# Autodesk Inventor assembly: link_first
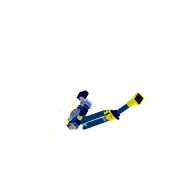
[picture p0: Inventor's stored thumbnail of the model, 180x180]
Saved by Autodesk Inventor 2020.5 (Build 245400000, 400)
## iProperties
Created: 2022-10-31
Part Number: link_first
Document SubType Name: Assembly
Designer: kanazawakotaro
Author: Administrator
## Documents named in this file (18)
- C:\Users\Administrator\Documents\kamuy2\kamuy2\link_first.iam
- C:\Users\Administrator\Documents\kamuy2\kamuy2\Parts\Part2_MIR_CPY_MIR.ipt
- C:\Users\Administrator\Documents\kamuy2\kamuy2\Parts\x-540_idle_MIR_CPY_MIR.ipt
- C:\Users\Administrator\Documents\kamuy2\kamuy2\Parts\GEABP1.0-32-10-A-12-KFC22-K3_Autodesk_Inventor_2020_20221101\AIS2020\GEABP1_0-32-10-A-12-KFC22-K3_MIR_CPY_MIR.iam
- C:\Users\Administrator\Documents\kamuy2\kamuy2\Parts\GEYK1.0-70-10-B-10K_Autodesk_Inventor_2020_20221114\AIS2020\GEYK1_0-70-10-B-10K_MIR_CPY_MIR.iam
- C:\Users\Administrator\Documents\kamuy2\kamuy2\Part16_MIR_CPY_MIR.ipt
- C:\Users\Administrator\Documents\kamuy2\kamuy2\Part1_MIR_CPY_MIR.ipt
- C:\Users\Administrator\Documents\kamuy2\kamuy2\Part13_MIR_CPY_MIR.ipt
- C:\Users\Administrator\Documents\kamuy2\kamuy2\Part17_MIR_CPY_MIR.ipt
- C:\Users\Administrator\Documents\kamuy2\kamuy2\Parts\SMYHF10_STEP_AP203AP214\SMYHF10_203_MIR_CPY_MIR.ipt
- C:\Users\Administrator\Documents\kamuy2\kamuy2\Parts\BGHK6800VV-30_Autodesk_Inventor_2020_20221102\AIS2020\BGHK6800VV-30_MIR_CPY_MIR.iam
- C:\Users\Administrator\Documents\kamuy2\kamuy2\Parts\XW540.N105.I101_MIR_CPY_MIR.ipt
- C:\Users\Administrator\Documents\kamuy2\kamuy2\Parts\NSFMKR10-67-KA22-A20_Autodesk_Inventor_2020_20221116\AIS2020\NSFMKR10-67-KA22-A20_MIR_CPY_MIR.iam
- C:\Users\Administrator\Documents\kamuy2\kamuy2\Parts\NSFMR10-37_Autodesk_Inventor_2020_20221116\AIS2020\NSFMR10-37(000_000)_MIR_CPY_MIR.iam
- C:\Users\Administrator\Documents\kamuy2\kamuy2\Parts\NSFMKRRA10-144-F3-S6-KA5-A18-KB108.5-B11_Autodesk_Inventor_2020_20221117\AIS2020\NSFMKRRA10-144-F3-S6-KA5-A18-KB108_5-B11_MIR_CPY_MIR.iam
- C:\Users\Administrator\Documents\kamuy2\kamuy2\LEG_MIR_MIR1_MIR.iam
- C:\Users\Administrator\Documents\foot3d.ipt
- C:\Users\Administrator\Documents\gom.ipt
## Components (27 placed, 17 different names)
1. Part2_MIR_CPY_MIR:1
2. x-540_idle_MIR_CPY_MIR:1 — メイト:51, メイト:50, フラッシュ:68, フラッシュ:66, フラッシュ:58, メイト:166, フラッシュ:103, メイト:256, メイト:39
3. GEABP1_0-32-10-A-12-KFC22-K3_MIR_CPY_MIR:1 [sub-assembly] — メイト:51, メイト:50, フラッシュ:20
4. GEYK1_0-70-10-B-10K_MIR_CPY_MIR:1 [sub-assembly] — フラッシュ:61, フラッシュ:136, メイト:248
5. x-540_idle_MIR_CPY_MIR:2 — フラッシュ:68, フラッシュ:66, フラッシュ:58, メイト:86, メイト:85, フラッシュ:100, メイト:183, メイト:180, メイト:179, メイト:178
6. GEABP1_0-32-10-A-12-KFC22-K3_MIR_CPY_MIR:2 [sub-assembly] — フラッシュ:61, メイト:86, メイト:85
7. Part16_MIR_CPY_MIR:1 — メイト:170
8. Part16_MIR_CPY_MIR:2 — メイト:171
9. Part1_MIR_CPY_MIR:1 — メイト:171, フラッシュ:100
10. Part1_MIR_CPY_MIR:2 — メイト:183, メイト:170, メイト:166, メイト:38, メイト:39
11. Part13_MIR_CPY_MIR:1 — フラッシュ:103, フラッシュ:108, フラッシュ:104, メイト:172, メイト:208
12. Part17_MIR_CPY_MIR:1 — フラッシュ:108, フラッシュ:104, メイト:172, フラッシュ:105, メイト:174, メイト:177
13. SMYHF10_203_MIR_CPY_MIR:1 — フラッシュ:105, メイト:174, メイト:254
14. GEYK1_0-70-10-B-10K_MIR_CPY_MIR:2 [sub-assembly] — メイト:177, メイト:65, メイト:207
15. Part13_MIR_CPY_MIR:2 — メイト:180, メイト:179, メイト:178, フラッシュ:110, メイト:194, メイト:214
16. SMYHF10_203_MIR_CPY_MIR:2 — メイト:187, メイト:185, メイト:213
17. Part17_MIR_CPY_MIR:2 — フラッシュ:110, メイト:194, メイト:187, メイト:185, メイト:211, メイト:215
18. BGHK6800VV-30_MIR_CPY_MIR:1 [sub-assembly] — メイト:65, フラッシュ:33, フラッシュ:32, メイト:205, メイト:209, フラッシュ:116, フラッシュ:115
19. GEABP1_0-32-10-A-12-KFC22-K3_MIR_CPY_MIR:3 [sub-assembly] — メイト:204, メイト:203
20. XW540.N105.I101_MIR_CPY_MIR:1 — フラッシュ:33, フラッシュ:32, メイト:205, メイト:204, メイト:203
21. NSFMKR10-67-KA22-A20_MIR_CPY_MIR:1 [sub-assembly] — メイト:254, メイト:209, メイト:208, メイト:207
22. BGHK6800VV-30_MIR_CPY_MIR:2 [sub-assembly] — メイト:211, フラッシュ:116, フラッシュ:115, メイト:212
23. NSFMR10-37(000_000)_MIR_CPY_MIR:1 [sub-assembly] — メイト:215, メイト:214, メイト:213, メイト:212
24. NSFMKRRA10-144-F3-S6-KA5-A18-KB108_5-B11_MIR_CPY_MIR:1 [sub-assembly] — メイト:256, フラッシュ:136, メイト:248, メイト:37, メイト:38
25. LEG_MIR_MIR1_MIR:1 [sub-assembly] — メイト:37, フラッシュ:20, メイト:42, メイト:43, フラッシュ:22
26. foot3d:1 — メイト:42, メイト:43, フラッシュ:22
27. gom:1
## Relationships (57: Mate 39, Flush 18)
- メイト:51 [Mate]: x-540_idle_MIR_CPY_MIR:1 ↔ GEABP1_0-32-10-A-12-KFC22-K3_MIR_CPY_MIR:1
- メイト:50 [Mate] (4 mm): x-540_idle_MIR_CPY_MIR:1 ↔ GEABP1_0-32-10-A-12-KFC22-K3_MIR_CPY_MIR:1
- フラッシュ:68 [Flush]: x-540_idle_MIR_CPY_MIR:1 ↔ x-540_idle_MIR_CPY_MIR:2
- フラッシュ:66 [Flush]: x-540_idle_MIR_CPY_MIR:1 ↔ x-540_idle_MIR_CPY_MIR:2
- フラッシュ:58 [Flush]: x-540_idle_MIR_CPY_MIR:1 ↔ x-540_idle_MIR_CPY_MIR:2
- フラッシュ:61 [Flush]: GEYK1_0-70-10-B-10K_MIR_CPY_MIR:1 ↔ GEABP1_0-32-10-A-12-KFC22-K3_MIR_CPY_MIR:2
- メイト:86 [Mate] (4 mm): x-540_idle_MIR_CPY_MIR:2 ↔ GEABP1_0-32-10-A-12-KFC22-K3_MIR_CPY_MIR:2
- メイト:85 [Mate]: x-540_idle_MIR_CPY_MIR:2 ↔ GEABP1_0-32-10-A-12-KFC22-K3_MIR_CPY_MIR:2
- メイト:171 [Mate]: Part16_MIR_CPY_MIR:2 ↔ Part1_MIR_CPY_MIR:1
- フラッシュ:100 [Flush]: x-540_idle_MIR_CPY_MIR:2 ↔ Part1_MIR_CPY_MIR:1
- メイト:183 [Mate]: x-540_idle_MIR_CPY_MIR:2 ↔ Part1_MIR_CPY_MIR:2
- メイト:170 [Mate]: Part16_MIR_CPY_MIR:1 ↔ Part1_MIR_CPY_MIR:2
- メイト:166 [Mate]: x-540_idle_MIR_CPY_MIR:1 ↔ Part1_MIR_CPY_MIR:2
- フラッシュ:103 [Flush]: x-540_idle_MIR_CPY_MIR:1 ↔ Part13_MIR_CPY_MIR:1
- フラッシュ:108 [Flush]: Part13_MIR_CPY_MIR:1 ↔ Part17_MIR_CPY_MIR:1
- フラッシュ:104 [Flush]: Part13_MIR_CPY_MIR:1 ↔ Part17_MIR_CPY_MIR:1
- メイト:172 [Mate] (15 mm): Part13_MIR_CPY_MIR:1 ↔ Part17_MIR_CPY_MIR:1
- フラッシュ:105 [Flush] (0.1 mm): Part17_MIR_CPY_MIR:1 ↔ SMYHF10_203_MIR_CPY_MIR:1
- メイト:174 [Mate]: Part17_MIR_CPY_MIR:1 ↔ SMYHF10_203_MIR_CPY_MIR:1
- メイト:177 [Mate] (5 mm): Part17_MIR_CPY_MIR:1 ↔ GEYK1_0-70-10-B-10K_MIR_CPY_MIR:2
- メイト:180 [Mate]: x-540_idle_MIR_CPY_MIR:2 ↔ Part13_MIR_CPY_MIR:2
- メイト:179 [Mate]: x-540_idle_MIR_CPY_MIR:2 ↔ Part13_MIR_CPY_MIR:2
- メイト:178 [Mate]: x-540_idle_MIR_CPY_MIR:2 ↔ Part13_MIR_CPY_MIR:2
- フラッシュ:110 [Flush]: Part13_MIR_CPY_MIR:2 ↔ Part17_MIR_CPY_MIR:2
- メイト:194 [Mate] (15 mm): Part13_MIR_CPY_MIR:2 ↔ Part17_MIR_CPY_MIR:2
- メイト:187 [Mate]: SMYHF10_203_MIR_CPY_MIR:2 ↔ Part17_MIR_CPY_MIR:2
- メイト:185 [Mate]: SMYHF10_203_MIR_CPY_MIR:2 ↔ Part17_MIR_CPY_MIR:2
- メイト:65 [Mate] (4 mm): GEYK1_0-70-10-B-10K_MIR_CPY_MIR:2 ↔ BGHK6800VV-30_MIR_CPY_MIR:1
- フラッシュ:33 [Flush]: BGHK6800VV-30_MIR_CPY_MIR:1 ↔ XW540.N105.I101_MIR_CPY_MIR:1
- フラッシュ:32 [Flush]: BGHK6800VV-30_MIR_CPY_MIR:1 ↔ XW540.N105.I101_MIR_CPY_MIR:1
- メイト:205 [Mate] (6.591 mm): BGHK6800VV-30_MIR_CPY_MIR:1 ↔ XW540.N105.I101_MIR_CPY_MIR:1
- メイト:204 [Mate]: GEABP1_0-32-10-A-12-KFC22-K3_MIR_CPY_MIR:3 ↔ XW540.N105.I101_MIR_CPY_MIR:1
- メイト:203 [Mate]: GEABP1_0-32-10-A-12-KFC22-K3_MIR_CPY_MIR:3 ↔ XW540.N105.I101_MIR_CPY_MIR:1
- メイト:254 [Mate]: SMYHF10_203_MIR_CPY_MIR:1 ↔ NSFMKR10-67-KA22-A20_MIR_CPY_MIR:1
- メイト:209 [Mate]: BGHK6800VV-30_MIR_CPY_MIR:1 ↔ NSFMKR10-67-KA22-A20_MIR_CPY_MIR:1
- メイト:208 [Mate]: Part13_MIR_CPY_MIR:1 ↔ NSFMKR10-67-KA22-A20_MIR_CPY_MIR:1
- メイト:207 [Mate]: GEYK1_0-70-10-B-10K_MIR_CPY_MIR:2 ↔ NSFMKR10-67-KA22-A20_MIR_CPY_MIR:1
- メイト:211 [Mate] (4 mm): Part17_MIR_CPY_MIR:2 ↔ BGHK6800VV-30_MIR_CPY_MIR:2
- フラッシュ:116 [Flush]: BGHK6800VV-30_MIR_CPY_MIR:1 ↔ BGHK6800VV-30_MIR_CPY_MIR:2
- フラッシュ:115 [Flush]: BGHK6800VV-30_MIR_CPY_MIR:1 ↔ BGHK6800VV-30_MIR_CPY_MIR:2
- メイト:215 [Mate]: Part17_MIR_CPY_MIR:2 ↔ NSFMR10-37(000_000)_MIR_CPY_MIR:1
- メイト:214 [Mate]: Part13_MIR_CPY_MIR:2 ↔ NSFMR10-37(000_000)_MIR_CPY_MIR:1
- メイト:213 [Mate]: SMYHF10_203_MIR_CPY_MIR:2 ↔ NSFMR10-37(000_000)_MIR_CPY_MIR:1
- メイト:212 [Mate]: BGHK6800VV-30_MIR_CPY_MIR:2 ↔ NSFMR10-37(000_000)_MIR_CPY_MIR:1
- メイト:256 [Mate] (31.591 mm): x-540_idle_MIR_CPY_MIR:1 ↔ NSFMKRRA10-144-F3-S6-KA5-A18-KB108_5-B11_MIR_CPY_MIR:1
- フラッシュ:136 [Flush] (-3 mm): GEYK1_0-70-10-B-10K_MIR_CPY_MIR:1 ↔ NSFMKRRA10-144-F3-S6-KA5-A18-KB108_5-B11_MIR_CPY_MIR:1
- メイト:248 [Mate]: GEYK1_0-70-10-B-10K_MIR_CPY_MIR:1 ↔ NSFMKRRA10-144-F3-S6-KA5-A18-KB108_5-B11_MIR_CPY_MIR:1
- メイト:37 [Mate]: NSFMKRRA10-144-F3-S6-KA5-A18-KB108_5-B11_MIR_CPY_MIR:1 ↔ LEG_MIR_MIR1_MIR:1
- フラッシュ:20 [Flush]: GEABP1_0-32-10-A-12-KFC22-K3_MIR_CPY_MIR:1 ↔ LEG_MIR_MIR1_MIR:1
- メイト:38 [Mate]: Part1_MIR_CPY_MIR:2 ↔ NSFMKRRA10-144-F3-S6-KA5-A18-KB108_5-B11_MIR_CPY_MIR:1
- メイト:39 [Mate]: x-540_idle_MIR_CPY_MIR:1 ↔ Part1_MIR_CPY_MIR:2
- [Flush]: foot3d:1 ↔ gom:1
- [Mate]: foot3d:1 ↔ gom:1
- [Mate]: foot3d:1 ↔ gom:1
- メイト:42 [Mate]: LEG_MIR_MIR1_MIR:1 ↔ foot3d:1
- メイト:43 [Mate]: LEG_MIR_MIR1_MIR:1 ↔ foot3d:1
- フラッシュ:22 [Flush] (10 mm): LEG_MIR_MIR1_MIR:1 ↔ foot3d:1
